# Autodesk Inventor assembly: 12inlift
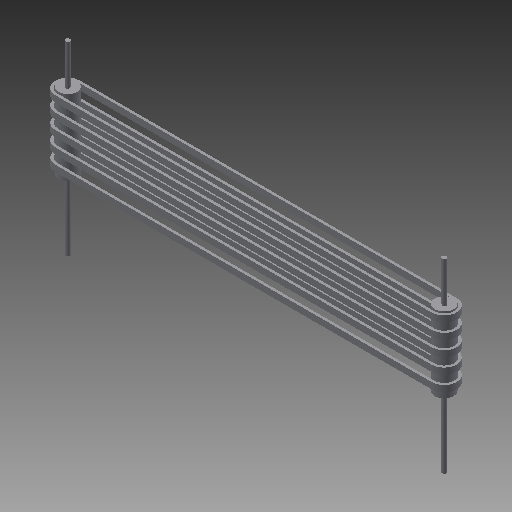
[picture p0: Inventor's stored thumbnail of the model, 512x512]
Saved by Autodesk Inventor 2017 (Build 210142000, 142)
## iProperties
Created: 2016-12-21
Part Number: 12inlift
Document SubType Name: Assembly
Designer: RoboticsUser
Author: RoboticsUser
## Documents named in this file (4)
- C:\Robotics\CAD\2016-17_CAD\12inlift.iam
- C:\Robotics\CAD\2016-17_CAD\LiftLine.ipt
- C:\Robotics\CAD\2016-17_CAD\4inax.ipt
- C:\Robotics\CAD\2016-17_CAD\16inchliftwire.ipt
## Components (9 placed, 3 different names)
1. LiftLine:1 — Mate:5, Insert:1, Insert:2, Insert:3, Insert:4, Insert:5, Flush:1
2. LiftLine:2 — Mate:4, Insert:6, Flush:2
3. 4inax:1 — Mate:4, Flush:2
4. 4inax:2 — Mate:5, Flush:1
5. 16inchliftwire:1 — Insert:5
6. 16inchliftwire:2 — Insert:4
7. 16inchliftwire:3 — Insert:3
8. 16inchliftwire:4 — Insert:2
9. 16inchliftwire:5 — Insert:1, Insert:6
## Relationships (10: Insert 6, Mate 2, Flush 2)
- Mate:4: LiftLine:2 ↔ 4inax:1
- Mate:5: LiftLine:1 ↔ 4inax:2
- Insert:1 (-7.62 mm): LiftLine:1 ↔ 16inchliftwire:5
- Insert:2 (-22.86 mm): LiftLine:1 ↔ 16inchliftwire:4
- Insert:3 (-38.1 mm): LiftLine:1 ↔ 16inchliftwire:3
- Insert:4 (-53.34 mm): LiftLine:1 ↔ 16inchliftwire:2
- Insert:5 (-68.58 mm): LiftLine:1 ↔ 16inchliftwire:1
- Insert:6 (-7.62 mm): LiftLine:2 ↔ 16inchliftwire:5
- Flush:1 (-40.64 mm): LiftLine:1 ↔ 4inax:2
- Flush:2 (-40.64 mm): LiftLine:2 ↔ 4inax:1
